# Autodesk Inventor assembly: Assembly1
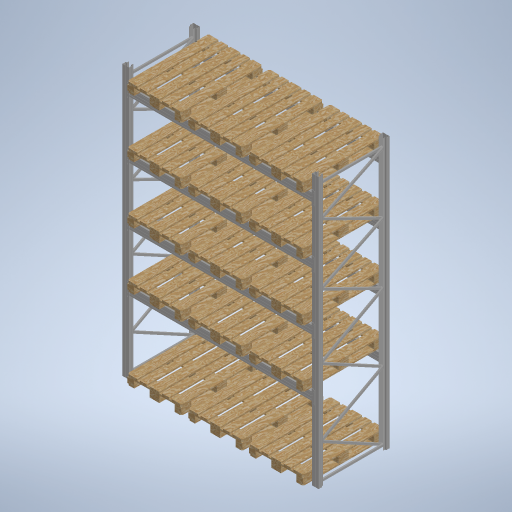
[picture p0: Inventor's stored thumbnail of the model, 512x512]
Saved by Autodesk Inventor 2024 (Build 280153000, 153)
## iProperties
Created: 2024-04-04
Part Number: Assembly1
Document SubType Name: Assembly
Designer: Gabek
Author: Gabek
## Documents named in this file (2)
- D:\factory-digital-twin\src\assets\glb_models\Assembly1.iam
- D:\glb_models\cad\heavy-rack-unit-1050x4000-1.snapshot.2\Heavy Rack 105x400_Simplify_1.ipt
## Components (1 placed, 1 different names)
1. Heavy Rack 105x400_Simplify_1:1 — Mate:1, Mate:2, Mate:3
## Relationships (3: Mate 3)
- Mate:1: Heavy Rack 105x400_Simplify_1:1
- Mate:2: Heavy Rack 105x400_Simplify_1:1
- Mate:3: Heavy Rack 105x400_Simplify_1:1
